# Autodesk Inventor assembly: CJ2KB10-60RZ(0_1_0)
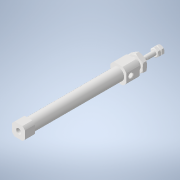
[picture p0: Inventor's stored thumbnail of the model, 180x180]
Saved by Autodesk Inventor 2022.3 (Build 263350000, 350)
## iProperties
Company: CADENAS
Created: 2022-05-15
Part Number: CJ2KB10-60RZ(0_1_0)
Description: STEP AP203
Document SubType Name: Assembly
Designer: YusukeKunita
Sending System: PARTsolutions
Title: e:/temp/worker_170/temp/exporttempdir_32_269_Bwl5F/format_0/CJ2KB10-60RZ(0_1_0).stp
Author: License CC BY-ND 4.0
Revision Number: NONE
## Documents named in this file (5)
- C:\Users\YusukeKunita\Documents\GrabCAD\Development\BasicParts\AirCylinder\CJ2KB10-60RZ\CJ2KB10-60RZ.iam
- C:\Users\YusukeKunita\Documents\GrabCAD\Development\BasicParts\AirCylinder\CJ2KB10-60RZ\CJ2KB10-60RZ_BODY.ipt
- C:\Users\YusukeKunita\Documents\GrabCAD\Development\BasicParts\AirCylinder\CJ2KB10-60RZ\CJ2K10Z_NUT.ipt
- C:\Users\YusukeKunita\Documents\GrabCAD\Development\BasicParts\AirCylinder\CJ2KB10-60RZ\CJ2KB10-60Z_ROD.ipt
- C:\Users\YusukeKunita\Documents\GrabCAD\Development\BasicParts\AirCylinder\CJ2KB10-60RZ\NTJ-010C.ipt
## Components (5 placed, 5 different names)
1. NAUO1 — フラッシュ:1, 円柱状:1, 回転:1
2. NAUO2 — 回転:1
3. NAUO3 — フラッシュ:1, 円柱状:1, 回転:2
4. NAUO4 — 回転:3
5. NAUO5 — 回転:2, 回転:3
## Relationships (5: RevoluteJoint 3, Flush 1, CylindricalJoint 1)
- フラッシュ:1 [Flush] (20 mm): NAUO1 ↔ NAUO3
- 円柱状:1 [CylindricalJoint]: NAUO1 ↔ NAUO3
- 回転:1 [RevoluteJoint]: NAUO1 ↔ NAUO2
- 回転:2 [RevoluteJoint]: NAUO3 ↔ NAUO5
- 回転:3 [RevoluteJoint]: NAUO4 ↔ NAUO5
